# Autodesk Inventor assembly: Assembly
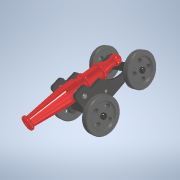
[picture p0: Inventor's stored thumbnail of the model, 180x180]
Saved by Autodesk Inventor 2022.2 (Build 262287000, 287)
## iProperties
Created: 2022-02-03
Part Number: Assembly
Document SubType Name: Assembly
Designer: PRASHANTH
Author: PRASHANTH
## Documents named in this file (7)
- E:\BME\Autodesk Sample\Assembly.iam
- E:\BME\Autodesk Sample\IPT Files\Cannon.ipt
- E:\BME\Autodesk Sample\IPT Files\Side.ipt
- E:\BME\Autodesk Sample\IPT Files\Wheel_axle.ipt
- E:\BME\Autodesk Sample\IPT Files\Cannon_pin.ipt
- E:\BME\Autodesk Sample\IPT Files\Cannon_support_pin.ipt
- E:\BME\Autodesk Sample\IPT Files\Wheel.ipt
## Components (11 placed, 6 different names)
1. Side:1 — Mate:5, Mate:6, Mate:7, Mate:10, Flush:1, Mate:11, Mate:14, Flush:2
2. Side:2 — Mate:1, Mate:2, Mate:3, Mate:4, Mate:8, Mate:9, Mate:16, Mate:18
3. Wheel_axle:1 — Mate:2, Mate:3, Mate:5, Mate:12, Mate:17
4. Wheel_axle:2 — Mate:1, Mate:4, Mate:6, Mate:7, Mate:13, Mate:15, Tangent:1
5. Cannon_pin:1 — Mate:8, Mate:9, Mate:19
6. Cannon_support_pin:1 — Mate:10, Flush:1
7. Wheel:1 — Mate:17, Mate:18
8. Wheel:2 — Mate:15, Mate:16
9. Wheel:3 — Mate:11, Mate:12
10. Wheel:4 — Mate:13, Mate:14
11. Cannon:1 — Mate:19, Flush:2, Tangent:1
## Relationships (22: Mate 19, Flush 2, Tangent 1)
- Mate:1: Side:2 ↔ Wheel_axle:2
- Mate:2: Side:2 ↔ Wheel_axle:1
- Mate:3: Side:2 ↔ Wheel_axle:1
- Mate:4: Side:2 ↔ Wheel_axle:2
- Mate:5: Side:1 ↔ Wheel_axle:1
- Mate:6: Side:1 ↔ Wheel_axle:2
- Mate:7: Side:1 ↔ Wheel_axle:2
- Mate:8: Side:2 ↔ Cannon_pin:1
- Mate:9: Side:2 ↔ Cannon_pin:1
- Mate:10: Side:1 ↔ Cannon_support_pin:1
- Flush:1: Side:1 ↔ Cannon_support_pin:1
- Mate:11 (2 mm): Side:1 ↔ Wheel:3
- Mate:12: Wheel_axle:1 ↔ Wheel:3
- Mate:13: Wheel_axle:2 ↔ Wheel:4
- Mate:14 (2 mm): Side:1 ↔ Wheel:4
- Mate:15: Wheel_axle:2 ↔ Wheel:2
- Mate:16 (2 mm): Side:2 ↔ Wheel:2
- Mate:17: Wheel_axle:1 ↔ Wheel:1
- Mate:18 (2 mm): Side:2 ↔ Wheel:1
- Mate:19: Cannon_pin:1 ↔ Cannon:1
- Flush:2 (-21.9964 mm): Side:1 ↔ Cannon:1
- Tangent:1: Wheel_axle:2 ↔ Cannon:1
